# Autodesk Inventor assembly: alojamento_sensor_temperatura
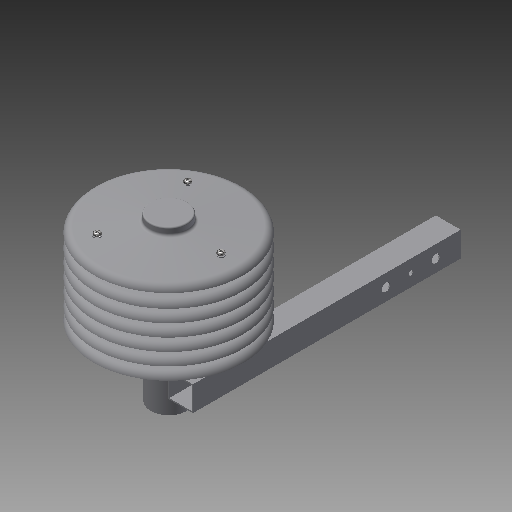
[picture p0: Inventor's stored thumbnail of the model, 512x512]
Saved by Autodesk Inventor 2019.4 (Build 234330000, 330)
## iProperties
Created: 2021-02-17
Part Number: alojamento_sensor_temperatura
Material: Genérico
Document SubType Name: Assembly
Designer: Lattes
Author: Lattes
## Documents named in this file (6)
- C:\Users\Lattes\Documents\GitHub\estacao-meteorologica\Estrutura\inventor\estrutura versão remota\Alojamento do Sensor de Temperatura e Umidade\alojamento_sensor_temperatura.iam
- C:\Users\Lattes\Documents\GitHub\estacao-meteorologica\Estrutura\inventor\estrutura versão remota\Alojamento do Sensor de Temperatura e Umidade\internas.ipt
- C:\Users\Lattes\Documents\GitHub\estacao-meteorologica\Estrutura\inventor\estrutura versão remota\Alojamento do Sensor de Temperatura e Umidade\tampa.ipt
- C:\Users\Lattes\Documents\GitHub\estacao-meteorologica\Estrutura\inventor\estrutura versão remota\Alojamento do Sensor de Temperatura e Umidade\Parafuso m3 70mm.ipt
- C:\Users\Lattes\Documents\GitHub\estacao-meteorologica\Estrutura\inventor\estrutura versão remota\Alojamento do Sensor de Temperatura e Umidade\porca m3.ipt
- C:\Users\Lattes\Documents\GitHub\estacao-meteorologica\Estrutura\inventor\estrutura versão remota\Alojamento do Sensor de Temperatura e Umidade\base e suporte.ipt
## Components (14 placed, 5 different names)
1. internas:1 — Inserir:1, Inserir:10, Inserir:11, Inserir:12, Inserir:13
2. internas:2 — Inserir:1, Inserir:2
3. internas:3 — Inserir:2, Inserir:3
4. internas:4 — Inserir:3, Inserir:4
5. internas:5 — Inserir:4, Inserir:5
6. internas:6 — Inserir:5, Inserir:6
7. tampa:1 — Inserir:6, Inserir:7, Inserir:8, Inserir:9
8. Parafuso m3 70mm:1 — Inserir:8
9. Parafuso m3 70mm:2 — Inserir:9
10. Parafuso m3 70mm:3 — Inserir:7
11. porca m3:1 — Inserir:12
12. porca m3:2 — Inserir:11
13. porca m3:3 — Inserir:10
14. base e suporte:1 — Inserir:13
## Relationships (13: Insert 13)
- Inserir:1: internas:1 ↔ internas:2
- Inserir:2: internas:2 ↔ internas:3
- Inserir:3: internas:3 ↔ internas:4
- Inserir:4: internas:4 ↔ internas:5
- Inserir:5: internas:5 ↔ internas:6
- Inserir:6: internas:6 ↔ tampa:1
- Inserir:7: tampa:1 ↔ Parafuso m3 70mm:3
- Inserir:8: tampa:1 ↔ Parafuso m3 70mm:1
- Inserir:9: tampa:1 ↔ Parafuso m3 70mm:2
- Inserir:10: internas:1 ↔ porca m3:3
- Inserir:11: internas:1 ↔ porca m3:2
- Inserir:12: internas:1 ↔ porca m3:1
- Inserir:13: internas:1 ↔ base e suporte:1
